# Autodesk Inventor assembly: nanopc_t4
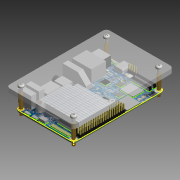
[picture p0: Inventor's stored thumbnail of the model, 180x180]
Saved by Autodesk Inventor 2013 SP2 (Build 170200200, 200)
## iProperties
Created: 2018-09-03
Part Number: nanopc_t4
Document SubType Name: Assembly
Designer: alex
Author: alex
## Documents named in this file (13)
- Z:\cluster-coffer\hardware\nanopc_t4\3d\nanopc_t4.iam
- Z:\cluster-coffer\hardware\nanopc_t4\3d\nanopc_t4_board.ipt
- Z:\cluster-coffer\hardware\nanopc_t4\3d\nanopc_t4_pin.ipt
- Z:\cluster-coffer\hardware\nanopc_t4\3d\nanopc_t4_rj45.ipt
- Z:\cluster-coffer\hardware\nanopc_t4\3d\nanopc_t4_usb3.ipt
- Z:\cluster-coffer\hardware\nanopc_t4\3d\nanopc_t4_headphone.ipt
- Z:\cluster-coffer\hardware\nanopc_t4\3d\nanopc_t4_usb.ipt
- Z:\cluster-coffer\hardware\nanopc_t4\3d\nanopc_t4_hdmi.ipt
- Z:\cluster-coffer\hardware\nanopc_t4\3d\nanopc_t4_pwr.ipt
- Z:\cluster-coffer\hardware\nanopc_t4\3d\nanopc_t4_usb3c.ipt
- Z:\cluster-coffer\hardware\nanopc_t4\3d\nanopc_t4_spacer_long.ipt
- Z:\cluster-coffer\hardware\nanopc_t4\3d\nanopc_t4_cover.ipt
- C:\Users\alex\Documents\Inventor\Content Center Files\R2013\en-US\ANSI B18.6.7M(00)\ANSI B18.6.7M - M3x0.5 x 8(4).ipt
## Components (67 placed, 12 different names)
1. nanopc_t4_board:1 — Mate:1, Mate:2, Mate:4, Flush:1, Flush:2, Flush:3, Flush:4, Flush:5, Flush:6, Flush:7, Flush:8, Mate:5, Flush:9, Flush:10, Flush:11, Flush:12, Flush:13, Flush:14, Flush:15, Flush:16, Flush:17, Insert:1, Insert:2, Insert:3
2. nanopc_t4_rj45:1 — Flush:1, Flush:2
3. nanopc_t4_usb3:1 — Flush:3, Flush:4
4. nanopc_t4_headphone:1 — Flush:5, Flush:6
5. nanopc_t4_usb:1 — Flush:7, Flush:8, Mate:6, Mate:7
6. nanopc_t4_usb:2 — Mate:5, Mate:6, Mate:7
7. nanopc_t4_hdmi:1 — Flush:9, Flush:10, Flush:11
8. nanopc_t4_pwr:1 — Flush:12, Flush:13
9. nanopc_t4_usb3c:1 — Flush:14, Flush:15
10. nanopc_t4_spacer_long:1 — Flush:16, Flush:17
11. nanopc_t4_spacer_long:2 — Insert:2
12. nanopc_t4_spacer_long:3 — Insert:3
13. nanopc_t4_spacer_long:4 — Insert:1
14. nanopc_t4_cover:1 — Insert:4, Insert:5, Insert:6, Insert:7
15. Cross Recessed Pan Head Machine Screw - Type I - Metric M3x0.5 x 8:1 — Insert:4
16. Cross Recessed Pan Head Machine Screw - Type I - Metric M3x0.5 x 8:2 — Insert:5
17. Cross Recessed Pan Head Machine Screw - Type I - Metric M3x0.5 x 8:3 — Insert:6
18. Cross Recessed Pan Head Machine Screw - Type I - Metric M3x0.5 x 8:4 — Insert:7
19. nanopc_t4_pin:1 — Mate:1, Mate:3, Mate:8
20. nanopc_t4_pin:2
21. nanopc_t4_pin:3
22. nanopc_t4_pin:4
23. nanopc_t4_pin:5
24. nanopc_t4_pin:6
25. nanopc_t4_pin:7
26. nanopc_t4_pin:8
27. nanopc_t4_pin:9
28. nanopc_t4_pin:10
29. nanopc_t4_pin:11
30. nanopc_t4_pin:12
31. nanopc_t4_pin:13
32. nanopc_t4_pin:14
33. nanopc_t4_pin:15
34. nanopc_t4_pin:16
35. nanopc_t4_pin:17
36. nanopc_t4_pin:18
37. nanopc_t4_pin:19
38. nanopc_t4_pin:20
39. nanopc_t4_pin:21
40. nanopc_t4_pin:22
41. nanopc_t4_pin:23
42. nanopc_t4_pin:24
43. nanopc_t4_pin:25
44. nanopc_t4_pin:26
45. nanopc_t4_pin:27
46. nanopc_t4_pin:28
47. nanopc_t4_pin:29
48. nanopc_t4_pin:30
49. nanopc_t4_pin:31
50. nanopc_t4_pin:32
51. nanopc_t4_pin:33
52. nanopc_t4_pin:34
53. nanopc_t4_pin:35
54. nanopc_t4_pin:36
55. nanopc_t4_pin:37
56. nanopc_t4_pin:38
57. nanopc_t4_pin:39
58. nanopc_t4_pin:40
59. nanopc_t4_pin:41 — Mate:2, Mate:3, Mate:8
60. nanopc_t4_pin:42
61. nanopc_t4_pin:43
62. nanopc_t4_pin:44
63. nanopc_t4_pin:45
64. nanopc_t4_pin:46 — Mate:4
65. nanopc_t4_pin:47
66. nanopc_t4_pin:48
67. nanopc_t4_pin:49
## Component patterns: (40 elements, first: nanopc_t4_pin:1), (5 elements, first: nanopc_t4_pin:41), (4 elements, first: nanopc_t4_pin:46)
## Relationships (32: Flush 17, Mate 8, Insert 7)
- Mate:1: nanopc_t4_board:1 ↔ nanopc_t4_pin:1
- Mate:2: nanopc_t4_board:1 ↔ nanopc_t4_pin:41
- Mate:3: nanopc_t4_pin:1 ↔ nanopc_t4_pin:41
- Mate:4: nanopc_t4_board:1 ↔ nanopc_t4_pin:46
- Flush:1: nanopc_t4_board:1 ↔ nanopc_t4_rj45:1
- Flush:2: nanopc_t4_board:1 ↔ nanopc_t4_rj45:1
- Flush:3: nanopc_t4_board:1 ↔ nanopc_t4_usb3:1
- Flush:4: nanopc_t4_board:1 ↔ nanopc_t4_usb3:1
- Flush:5: nanopc_t4_board:1 ↔ nanopc_t4_headphone:1
- Flush:6: nanopc_t4_board:1 ↔ nanopc_t4_headphone:1
- Flush:7: nanopc_t4_board:1 ↔ nanopc_t4_usb:1
- Flush:8: nanopc_t4_board:1 ↔ nanopc_t4_usb:1
- Mate:5: nanopc_t4_board:1 ↔ nanopc_t4_usb:2
- Mate:6: nanopc_t4_usb:1 ↔ nanopc_t4_usb:2
- Mate:7 (2.9 mm): nanopc_t4_usb:1 ↔ nanopc_t4_usb:2
- Mate:8: nanopc_t4_pin:1 ↔ nanopc_t4_pin:41
- Flush:9: nanopc_t4_board:1 ↔ nanopc_t4_hdmi:1
- Flush:10: nanopc_t4_board:1 ↔ nanopc_t4_hdmi:1
- Flush:11: nanopc_t4_board:1 ↔ nanopc_t4_hdmi:1
- Flush:12: nanopc_t4_board:1 ↔ nanopc_t4_pwr:1
- Flush:13: nanopc_t4_board:1 ↔ nanopc_t4_pwr:1
- Flush:14: nanopc_t4_board:1 ↔ nanopc_t4_usb3c:1
- Flush:15: nanopc_t4_board:1 ↔ nanopc_t4_usb3c:1
- Flush:16: nanopc_t4_board:1 ↔ nanopc_t4_spacer_long:1
- Flush:17: nanopc_t4_board:1 ↔ nanopc_t4_spacer_long:1
- Insert:1: nanopc_t4_board:1 ↔ nanopc_t4_spacer_long:4
- Insert:2: nanopc_t4_board:1 ↔ nanopc_t4_spacer_long:2
- Insert:3: nanopc_t4_board:1 ↔ nanopc_t4_spacer_long:3
- Insert:4: nanopc_t4_cover:1 ↔ Cross Recessed Pan Head Machine Screw - Type I - Metric M3x0.5 x 8:1
- Insert:5: nanopc_t4_cover:1 ↔ Cross Recessed Pan Head Machine Screw - Type I - Metric M3x0.5 x 8:2
- Insert:6: nanopc_t4_cover:1 ↔ Cross Recessed Pan Head Machine Screw - Type I - Metric M3x0.5 x 8:3
- Insert:7: nanopc_t4_cover:1 ↔ Cross Recessed Pan Head Machine Screw - Type I - Metric M3x0.5 x 8:4
